# Autodesk Inventor assembly: main
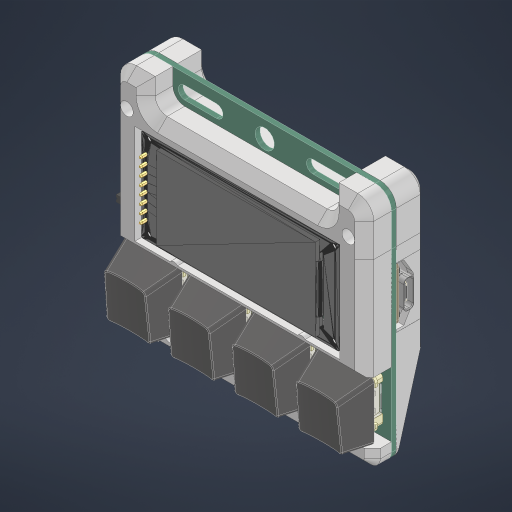
[picture p0: Inventor's stored thumbnail of the model, 512x512]
Saved by Autodesk Inventor 2024 (Build 280153000, 153)
## iProperties
Created: 2026-07-02
Part Number: main
Document SubType Name: Assembly
Designer: schar
Author: schar
## Documents named in this file (11)
- C:\Users\schar\Projects\Badge\foxbadge\cad\main.iam
- C:\Users\schar\Projects\Badge\foxbadge\cad\pcb\pcb.iam
- C:\Users\schar\Projects\Badge\foxbadge\cad\assets\low_profile_cherry_mx_asm.iam
- C:\Users\schar\Projects\Badge\foxbadge\cad\pcb\display\1.9inch-lcd-display.ipt
- C:\Users\schar\Projects\Badge\foxbadge\cad\pcb\display\1x8 Male Pin Header.ipt
- C:\Users\schar\Projects\Badge\foxbadge\cad\display_spacer.ipt
- C:\Users\schar\Projects\Badge\foxbadge\cad\screen_spacer_tube.ipt
- C:\Users\schar\Projects\Badge\foxbadge\cad\case_front.ipt
- C:\Users\schar\Projects\Badge\foxbadge\cad\front_case_buttons.ipt
- C:\Users\schar\Projects\Badge\foxbadge\cad\back_case.ipt
- C:\Users\schar\Projects\Badge\foxbadge\cad\pcb\pcb\XIAO-ESP32S3 v2\XIAO-ESP32S3 v2.iam
## Components (13 placed, 10 different names)
1. pcb:1 [sub-assembly] — Mate:1, Angle:1, Mate:2, Mate:3, Mate:4, Mate:5, Angle:2, Angle:3, Angle:4, Mate:6, Mate:7, Mate:8, Mate:12, Mate:15, Mate:24, Flush:4, Flush:5, Flush:6, Flush:7, Flush:8, Flush:9, Flush:10, Flush:11, Flush:12, Flush:14, Flush:15, Mate:26, Flush:16, Flush:17
2. low_profile_cherry_mx_asm:1 [sub-assembly] — Mate:1, Angle:1, Mate:2
3. low_profile_cherry_mx_asm:2 [sub-assembly] — Mate:3, Angle:2, Mate:8
4. low_profile_cherry_mx_asm:3 [sub-assembly] — Mate:4, Angle:3, Mate:7
5. low_profile_cherry_mx_asm:4 [sub-assembly] — Mate:5, Angle:4, Mate:6
6. 1.9inch-lcd-display:1 — Mate:18, Mate:23, Mate:25
7. 1x8 Male Pin Header:1 — Flush:1, Flush:2, Flush:3, Mate:24, Mate:25
8. display_spacer:1 — Flush:5, Flush:6, Flush:7
9. screen_spacer_tube:1 — Flush:8, Flush:9
10. case_front:1 — Flush:10, Flush:11, Flush:13
11. front_case_buttons:1 — Flush:12, Flush:13
12. back_case:1 — Flush:14, Flush:15
13. XIAO-ESP32S3 v2:1 [sub-assembly] — Mate:26, Flush:16, Flush:17
## Relationships (46: Mate 25, Flush 17, Angle 4)
- Mate:1: pcb:1 ↔ low_profile_cherry_mx_asm:1
- Angle:1 (0 deg): pcb:1 ↔ low_profile_cherry_mx_asm:1
- Mate:2: pcb:1 ↔ low_profile_cherry_mx_asm:1
- Mate:3: pcb:1 ↔ low_profile_cherry_mx_asm:2
- Mate:4: pcb:1 ↔ low_profile_cherry_mx_asm:3
- Mate:5: pcb:1 ↔ low_profile_cherry_mx_asm:4
- Angle:2 (0 deg): pcb:1 ↔ low_profile_cherry_mx_asm:2
- Angle:3 (0 deg): pcb:1 ↔ low_profile_cherry_mx_asm:3
- Angle:4 (0 deg): pcb:1 ↔ low_profile_cherry_mx_asm:4
- Mate:6: pcb:1 ↔ low_profile_cherry_mx_asm:4
- Mate:7: pcb:1 ↔ low_profile_cherry_mx_asm:3
- Mate:8: pcb:1 ↔ low_profile_cherry_mx_asm:2
- Flush:1 (-0.3 mm): 1x8 Male Pin Header:1
- Flush:2 (-0.3 mm): 1x8 Male Pin Header:1
- Mate:10
- Mate:11
- Flush:3 (-0.3 mm): 1x8 Male Pin Header:1
- Mate:12: pcb:1
- Mate:13
- Mate:14
- Mate:15: pcb:1
- Mate:16
- Mate:17
- Mate:18: 1.9inch-lcd-display:1
- Mate:19
- Mate:20
- Mate:21
- Mate:22
- Mate:23: 1.9inch-lcd-display:1
- Mate:24 (4 mm): pcb:1 ↔ 1x8 Male Pin Header:1
- Mate:25: 1.9inch-lcd-display:1 ↔ 1x8 Male Pin Header:1
- Flush:4: pcb:1
- Flush:5: pcb:1 ↔ display_spacer:1
- Flush:6: pcb:1 ↔ display_spacer:1
- Flush:7: pcb:1 ↔ display_spacer:1
- Flush:8: pcb:1 ↔ screen_spacer_tube:1
- Flush:9: pcb:1 ↔ screen_spacer_tube:1
- Flush:10: pcb:1 ↔ case_front:1
- Flush:11: pcb:1 ↔ case_front:1
- Flush:12: pcb:1 ↔ front_case_buttons:1
- Flush:13: case_front:1 ↔ front_case_buttons:1
- Flush:14: pcb:1 ↔ back_case:1
- Flush:15: pcb:1 ↔ back_case:1
- Mate:26: pcb:1 ↔ XIAO-ESP32S3 v2:1
- Flush:16 (0.46 mm): pcb:1 ↔ XIAO-ESP32S3 v2:1
- Flush:17 (20.108 mm): pcb:1 ↔ XIAO-ESP32S3 v2:1
